# Autodesk Inventor assembly: Table_Assembly
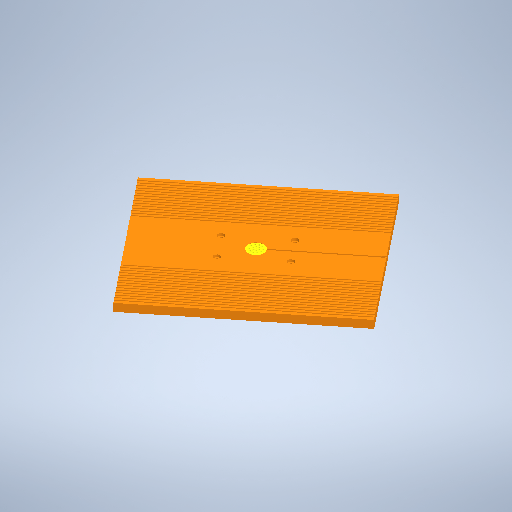
[picture p0: Inventor's stored thumbnail of the model, 512x512]
Saved by Autodesk Inventor 2025.2 (Build 292293000, 293)
## iProperties
Created: 2025-05-24
Part Number: Table_Assembly
Document SubType Name: Assembly
Designer: Musa Gamal
Author: Musa Gamal
## Documents named in this file (4)
- D:\ASU\senior 1\semster 2\Advanced Manufacturing Technology & Prototyping\Project\Table_Assembly.iam
- D:\ASU\senior 1\semster 2\Advanced Manufacturing Technology & Prototyping\Project\Filter_1.ipt
- D:\ASU\senior 1\semster 2\Advanced Manufacturing Technology & Prototyping\Project\Table_Filter.ipt
- D:\ASU\senior 1\semster 2\Advanced Manufacturing Technology & Prototyping\Project\Table_MU.ipt
## Components (3 placed, 3 different names)
1. Filter_1:1 — Mate:1, Mate:2
2. Table_Filter:1 — Mate:3, Mate:4, Mate:5
3. Table_MU:1 — Mate:1, Mate:2, Mate:3, Mate:4, Mate:5
## Relationships (5: Mate 5)
- Mate:1: Filter_1:1 ↔ Table_MU:1
- Mate:2: Filter_1:1 ↔ Table_MU:1
- Mate:3: Table_Filter:1 ↔ Table_MU:1
- Mate:4: Table_Filter:1 ↔ Table_MU:1
- Mate:5: Table_Filter:1 ↔ Table_MU:1
